# Autodesk Inventor assembly: Probe-clamp-v2
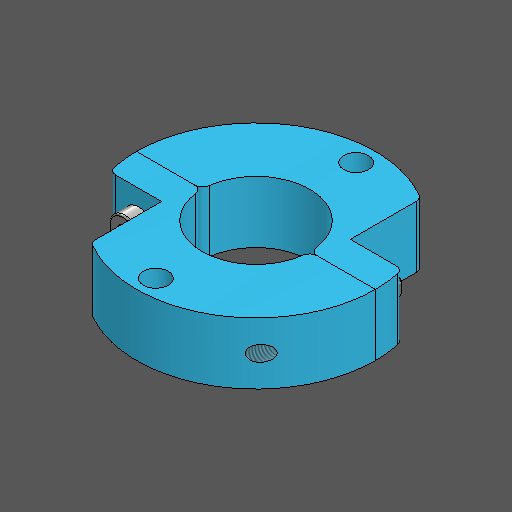
[picture p0: Inventor's stored thumbnail of the model, 512x512]
Saved by Autodesk Inventor 2025 (Build 290162000, 162)
## iProperties
Created: 2024-06-05
Part Number: Probe-clamp-v2
Document SubType Name: Assembly
Designer: kuzmin
Author: kuzmin
## Documents named in this file (4)
- C:\Users\queez\Dropbox\Drawings\PIHTI\PALP\Probe-clamp-v2.iam
- C:\Users\queez\Dropbox\Drawings\PIHTI\ContentCenter\Fastners\M2x8-SHCS.ipt
- C:\Users\queez\Dropbox\Drawings\PIHTI\PALP\WireHolderRing\WireHolderRing-ID14.ipt
- C:\Users\queez\Dropbox\Drawings\PIHTI\PALP\WireHolderRing.ipt
## Components (4 placed, 2 different names)
1. SS ISO 4762 M2 x 8:1
2. SS ISO 4762 M2 x 8:2
3. WireHolderRing-ID14:1
4. WireHolderRing-ID14:2
## Relationships (3: WeldJoint 2, Mate 1)
- [Mate]: WireHolderRing-ID14:1 ↔ WireHolderRing-ID14:2
- [WeldJoint]: SS ISO 4762 M2 x 8:2 ↔ WireHolderRing-ID14:2
- [WeldJoint]: SS ISO 4762 M2 x 8:1 ↔ WireHolderRing-ID14:1
